# Autodesk Inventor assembly: UNLHEP-13-01-A-009_StampStorage
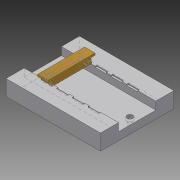
[picture p0: Inventor's stored thumbnail of the model, 180x180]
Saved by Autodesk Inventor 2013 (Build 170138000, 138)
## iProperties
Created: 2014-01-23
Part Number: UNLHEP-13-01-A-009_StampStorage
Document SubType Name: Assembly
Designer: Frank Meier
Author: Frank Meier
## Documents named in this file (3)
- C:\Users\Frank Meier\Documents\Inventor\Delvotec-Saugplatte\UNLHEP-14-01-A-009_StampStorage.iam
- C:\Users\Frank Meier\Documents\Inventor\Delvotec-Saugplatte\UNLHEP-14-01-P-016_StampStoragePlate.ipt
- C:\Users\Frank Meier\Documents\Inventor\Delvotec-Saugplatte\UNLHEP-14-01-A-006_Rubberstamp.iam
## Components (2 placed, 2 different names)
1. UNLHEP-14-01-P-016_StampStoragePlate:1 — Passend:1
2. UNLHEP-14-01-A-006_Rubberstamp:1 [sub-assembly] — Passend:1
## Relationships (1: Mate 1)
- Passend:1 [Mate]: UNLHEP-14-01-P-016_StampStoragePlate:1 ↔ UNLHEP-14-01-A-006_Rubberstamp:1
